# Autodesk Inventor assembly: Front_Upper_Arm_Assembly
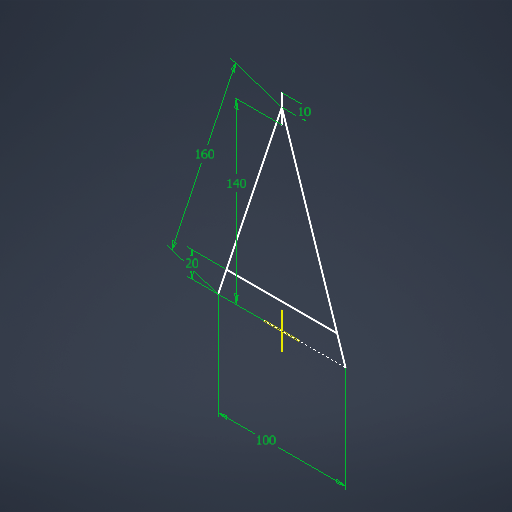
[picture p0: Inventor's stored thumbnail of the model, 512x512]
Saved by Autodesk Inventor 2026.1 (Build 301233000, 233)
## iProperties
Created: 2026-06-07
Part Number: Front_Upper_Arm_Assembly
Document SubType Name: Assembly
Designer: share
Author: share
## Documents named in this file (2)
- C:\Users\share\OneDrive\Documents\Personal Projects\GOGO Kart\CAD\GOGO_KART_FSAE\Shareef\Suspension Parts\Front Upper Arm\Front_Upper_Arm_Assembly.iam
- C:\Users\share\OneDrive\Documents\Personal Projects\GOGO Kart\CAD\GOGO_KART_FSAE\Shareef\Suspension Parts\Front Upper Arm\Front_Upper_Arm_Outline_Sketch.ipt
## Components (1 placed, 1 different names)
1. Front_Upper_Arm_Outline_Sketch:1 — Flush:1, Flush:2, Flush:3
## Relationships (3: Flush 3)
- Flush:1: Front_Upper_Arm_Outline_Sketch:1
- Flush:2: Front_Upper_Arm_Outline_Sketch:1
- Flush:3: Front_Upper_Arm_Outline_Sketch:1
